# Autodesk Inventor assembly: cylinder
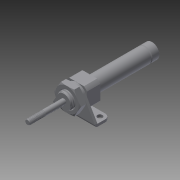
[picture p0: Inventor's stored thumbnail of the model, 180x180]
Saved by Autodesk Inventor 2013 (Build 170138000, 138)
## iProperties
Created: 2013-02-05
Part Number: cylinder
Document SubType Name: Assembly
Designer: Arpan
Author: Arpan
## Documents named in this file (3)
- C:\Users\Arpan\Documents\GitHub\frc2013CAD\Cimber actual\cylinder.iam
- C:\Users\Arpan\Documents\GitHub\frc2013CAD\Cimber actual\teensy weensy cylinder foot.ipt
- C:\Users\Arpan\Documents\GitHub\frc2013CAD\Cimber actual\small cylinder.ipt
## Components (2 placed, 2 different names)
1. teensy weensy cylinder foot:1 — Mate:1, Mate:2, Angle:1
2. small cylinder:1 — Mate:1, Mate:2, Angle:1
## Relationships (3: Mate 2, Angle 1)
- Mate:1: teensy weensy cylinder foot:1 ↔ small cylinder:1
- Mate:2: teensy weensy cylinder foot:1 ↔ small cylinder:1
- Angle:1 (0 deg): teensy weensy cylinder foot:1 ↔ small cylinder:1
